# Autodesk Inventor assembly: CandleHolder-Ocean
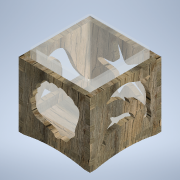
[picture p0: Inventor's stored thumbnail of the model, 180x180]
Saved by Autodesk Inventor 2021 (Build 250183000, 183)
## iProperties
Created: 2016-10-20
Part Number: CandleHolder-Ocean
Document SubType Name: Assembly
Designer: andrew
Author: andrew
## Documents named in this file (7)
- D:\Projects\cad_models\candle_holder\CandleHolder-Ocean.iam
- D:\Projects\cad_models\candle_holder\CandleHolder-1.ipt
- D:\Projects\cad_models\candle_holder\CandleHolder-Clam-14.ipt
- D:\Projects\cad_models\candle_holder\CandleHolder-Dolphin-13.ipt
- D:\Projects\cad_models\candle_holder\CandleHolder-Starfish-12.ipt
- D:\Projects\cad_models\candle_holder\CandleHolder-Wave-15.ipt
- D:\Projects\cad_models\candle_holder\CandleHolder-3.ipt
## Components (6 placed, 6 different names)
1. CandleHolder-1:1 — Mate:1, Mate:2, Flush:1, Mate:3, Mate:4, Mate:5, Mate:6, Flush:2, Flush:3, Flush:4, Flush:7, Mate:10
2. CandleHolder-Clam-14:1 — Mate:3, Flush:3, Flush:6
3. CandleHolder-Dolphin-13:1 — Mate:4, Flush:4, Mate:8
4. CandleHolder-Starfish-12:1 — Mate:5, Mate:9, Flush:7
5. CandleHolder-Wave-15:1 — Mate:6, Flush:2, Flush:5
6. CandleHolder-3:1 — Mate:10, Mate:11, Mate:12
## Relationships (18: Mate 11, Flush 7)
- Mate:1: CandleHolder-1:1
- Mate:2: CandleHolder-1:1
- Flush:1: CandleHolder-1:1
- Mate:3: CandleHolder-1:1 ↔ CandleHolder-Clam-14:1
- Mate:4: CandleHolder-1:1 ↔ CandleHolder-Dolphin-13:1
- Mate:5: CandleHolder-1:1 ↔ CandleHolder-Starfish-12:1
- Mate:6: CandleHolder-1:1 ↔ CandleHolder-Wave-15:1
- Flush:2 (6.35 mm): CandleHolder-1:1 ↔ CandleHolder-Wave-15:1
- Flush:3 (-6.35 mm): CandleHolder-1:1 ↔ CandleHolder-Clam-14:1
- Flush:4 (-6.35 mm): CandleHolder-1:1 ↔ CandleHolder-Dolphin-13:1
- Flush:5: CandleHolder-Wave-15:1
- Mate:8: CandleHolder-Dolphin-13:1
- Flush:6: CandleHolder-Clam-14:1
- Mate:9: CandleHolder-Starfish-12:1
- Flush:7 (6.35 mm): CandleHolder-1:1 ↔ CandleHolder-Starfish-12:1
- Mate:10: CandleHolder-1:1 ↔ CandleHolder-3:1
- Mate:11: CandleHolder-3:1
- Mate:12: CandleHolder-3:1
